# Autodesk Inventor assembly: Montagem_final
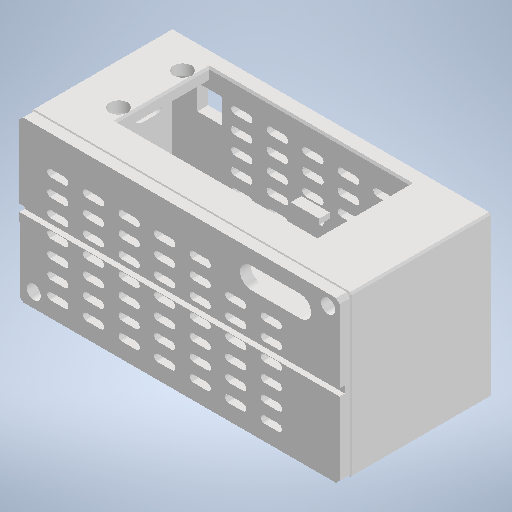
[picture p0: Inventor's stored thumbnail of the model, 512x512]
Saved by Autodesk Inventor 2025 (Build 290162000, 162)
## iProperties
Created: 2026-04-24
Part Number: Montagem_final
Document SubType Name: Assembly
Designer: pedro
Author: pedro
## Documents named in this file (3)
- C:\Users\pedro\OneDrive\Área de Trabalho\PEDRO\TCC - Eng. Controle e Automação\Prototipo peças\Prototipo Final\Montagem_final.iam
- C:\Users\pedro\OneDrive\Área de Trabalho\PEDRO\TCC - Eng. Controle e Automação\Prototipo peças\Prototipo Final\carcaça final.ipt
- C:\Users\pedro\OneDrive\Área de Trabalho\PEDRO\TCC - Eng. Controle e Automação\Prototipo peças\Prototipo Final\tampa final.ipt
## Components (2 placed, 2 different names)
1. carcaça final:1 — Inserir:1, Inserir:2, Inserir:3
2. tampa final:1 — Inserir:1, Inserir:2, Inserir:3
## Relationships (3: Insert 3)
- Inserir:1: carcaça final:1 ↔ tampa final:1
- Inserir:2: carcaça final:1 ↔ tampa final:1
- Inserir:3: carcaça final:1 ↔ tampa final:1
